# Autodesk Inventor assembly: SACMI DPA CARDBOARD POSITIONING SYSMEM_MIR
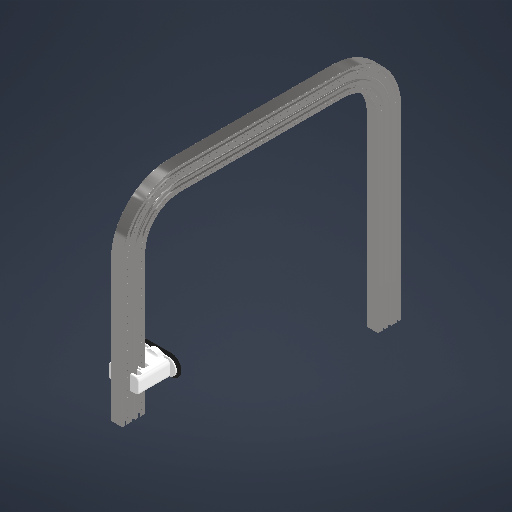
[picture p0: Inventor's stored thumbnail of the model, 512x512]
Saved by Autodesk Inventor 2025 (Build 290162000, 162)
## iProperties
Created: 2024-05-16
Part Number: SACMI DPA CARDBOARD POSITIONING SYSMEM_MIR
Document SubType Name: Assembly
Designer: zulet
Author: zulet
## Documents named in this file (3)
- D:\UNAL\2024-1S\APM\Digital Factory\Packaging Machine\SACMI DPA CARDBOARD POSITIONING SYSMEM_MIR.iam
- D:\UNAL\2024-1S\APM\Digital Factory\Packaging Machine\SACMI DPA C-RAIL_MIR.ipt
- D:\UNAL\2024-1S\APM\Digital Factory\Packaging Machine\SACMI DPA C-RAIL GRIP_MIR.ipt
## Components (2 placed, 2 different names)
1. SACMI DPA C-RAIL_MIR:1 — Flush:1, Flush:2, Mate:3
2. SACMI DPA C-RAIL GRIP_MIR:1 — Flush:1, Flush:2, Mate:3
## Relationships (3: Flush 3)
- Flush:1 (120 mm): SACMI DPA C-RAIL_MIR:1 ↔ SACMI DPA C-RAIL GRIP_MIR:1
- Flush:2: SACMI DPA C-RAIL_MIR:1 ↔ SACMI DPA C-RAIL GRIP_MIR:1
- Mate:3 [Flush]: SACMI DPA C-RAIL_MIR:1 ↔ SACMI DPA C-RAIL GRIP_MIR:1
